# Autodesk Inventor assembly: Alliance Short Mogo
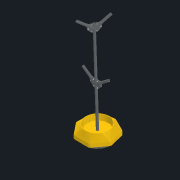
[picture p0: Inventor's stored thumbnail of the model, 180x180]
Saved by Autodesk Inventor 2021 (Build 250183000, 183)
## iProperties
Created: 2021-05-29
Part Number: Alliance Short Mogo
Document SubType Name: Assembly
Designer: max
Sending System: Autodesk Inventor 2021
Preprocessor: ST-DEVELOPER v18.1
Title: C:\Users\max\Desktop\Vex\TiP FieldCAD\Mogos\Alliance Short Mogo.stp
Author: max
Revision Number: ANY
## Documents named in this file (10)
- C:\Users\max\Desktop\Vex\TiP FieldCAD\Mogos\Alliance Tall Mogo.iam
- C:\Users\max\Desktop\Vex\TiP FieldCAD\Mogos\Screw 8-32 Steel .375.ipt
- C:\Users\max\Desktop\Vex\TiP FieldCAD\Mogos\Nut Nylock.ipt
- C:\Users\max\Desktop\Vex\TiP FieldCAD\Mogos\Mogo Branch Splitter.ipt
- C:\Users\max\Desktop\Vex\TiP FieldCAD\Mogos\Mogo Branch.ipt
- C:\Users\max\Desktop\Vex\TiP FieldCAD\Mogos\Mogo Post.ipt
- C:\Users\max\Desktop\Vex\TiP FieldCAD\Mogos\Mogo Base Post Grip.ipt
- C:\Users\max\Desktop\Vex\TiP FieldCAD\Mogos\Mogo Base Yellow.ipt
- C:\Users\max\Desktop\Vex\TiP FieldCAD\Mogos\Screw 8-32 Steel .625.ipt
- C:\Users\max\Desktop\Vex\TiP FieldCAD\Mogos\Mogo Base Bottom.ipt
## Components (45 placed, 9 different names)
1. Screw 8-32 Steel .375:1
2. Nut Nylock:1
3. Mogo Branch Splitter:1 — Angle:7
4. Mogo Branch:1
5. Mogo Post:1
6. Mogo Branch:2
7. Mogo Branch Splitter:2 — Mate:28, Mate:29
8. Screw 8-32 Steel .375:2
9. Nut Nylock:2
10. Screw 8-32 Steel .375:3
11. Nut Nylock:3
12. Screw 8-32 Steel .375:4
13. Nut Nylock:4
14. Screw 8-32 Steel .375:5
15. Nut Nylock:5
16. Screw 8-32 Steel .375:6
17. Nut Nylock:6
18. Mogo Base Post Grip:1
19. Mogo Base Yellow:1
20. Mogo Base Post Grip:2
21. Nut Nylock:7
22. Screw 8-32 Steel .625:7
23. Nut Nylock:8
24. Screw 8-32 Steel .625:8
25. Nut Nylock:9
26. Nut Nylock:10
27. Nut Nylock:11
28. Mogo Base Bottom:1
29. Mogo Branch Splitter:3 — Mate:8, Mate:9, Mate:10, Mate:11, Angle:7
30. Mogo Branch:3 — Mate:2, Mate:5
31. Mogo Post:2 — Mate:6, Mate:7, Mate:28, Mate:29
32. Mogo Branch:4 — Mate:3, Mate:4
33. Mogo Branch Splitter:4 — Mate:2, Mate:3, Mate:4, Mate:5, Mate:6, Mate:7, Mate:8, Mate:9, Mate:10, Mate:12, Mate:14, Mate:15, Mate:18, Mate:19, Mate:20, Mate:21, Mate:24, Mate:25, Angle:1, Angle:2, Mate:26, Mate:27, Angle:3, Angle:4, Angle:5, Angle:6
34. Screw 8-32 Steel .375:10 — Flush:1, Mate:1, Mate:11, Mate:12
35. Nut Nylock:15 — Flush:1, Mate:1, Angle:6
36. Screw 8-32 Steel .375:11 — Mate:14, Mate:15
37. Nut Nylock:16 — Angle:5
38. Screw 8-32 Steel .375:12 — Mate:18, Mate:20
39. Nut Nylock:17 — Angle:4
40. Screw 8-32 Steel .375:13 — Mate:19, Mate:21
41. Nut Nylock:18 — Angle:3
42. Screw 8-32 Steel .375:14 — Mate:26
43. Nut Nylock:19 — Mate:24, Angle:1
44. Screw 8-32 Steel .375:15 — Mate:27
45. Nut Nylock:20 — Mate:25, Angle:2
## Relationships (42: Mate 29, Angle 7, Flush 6)
- Flush:1 (-1.143 mm): Screw 8-32 Steel .375:10 ↔ Nut Nylock:15
- Mate:1: Screw 8-32 Steel .375:10 ↔ Nut Nylock:15
- Mate:2: Mogo Branch:3 ↔ Mogo Branch Splitter:4
- Mate:3: Mogo Branch:4 ↔ Mogo Branch Splitter:4
- Mate:4: Mogo Branch:4 ↔ Mogo Branch Splitter:4
- Mate:5: Mogo Branch:3 ↔ Mogo Branch Splitter:4
- Mate:6: Mogo Post:2 ↔ Mogo Branch Splitter:4
- Mate:7: Mogo Post:2 ↔ Mogo Branch Splitter:4
- Mate:8: Mogo Branch Splitter:3 ↔ Mogo Branch Splitter:4
- Mate:9: Mogo Branch Splitter:3 ↔ Mogo Branch Splitter:4
- Mate:10: Mogo Branch Splitter:3 ↔ Mogo Branch Splitter:4
- Mate:11: Mogo Branch Splitter:3 ↔ Screw 8-32 Steel .375:10
- Mate:12: Mogo Branch Splitter:4 ↔ Screw 8-32 Steel .375:10
- [Flush] (-1.143 mm): Screw 8-32 Steel .375:11 ↔ Nut Nylock:16
- [Mate]: Screw 8-32 Steel .375:11 ↔ Nut Nylock:16
- Mate:14: Mogo Branch Splitter:4 ↔ Screw 8-32 Steel .375:11
- Mate:15: Mogo Branch Splitter:4 ↔ Screw 8-32 Steel .375:11
- [Flush] (-1.143 mm): Screw 8-32 Steel .375:12 ↔ Nut Nylock:17
- [Mate]: Screw 8-32 Steel .375:12 ↔ Nut Nylock:17
- [Flush] (-1.143 mm): Screw 8-32 Steel .375:13 ↔ Nut Nylock:18
- [Mate]: Screw 8-32 Steel .375:13 ↔ Nut Nylock:18
- Mate:18: Mogo Branch Splitter:4 ↔ Screw 8-32 Steel .375:12
- Mate:19: Mogo Branch Splitter:4 ↔ Screw 8-32 Steel .375:13
- Mate:20: Mogo Branch Splitter:4 ↔ Screw 8-32 Steel .375:12
- Mate:21: Mogo Branch Splitter:4 ↔ Screw 8-32 Steel .375:13
- [Flush] (-1.143 mm): Screw 8-32 Steel .375:14 ↔ Nut Nylock:19
- [Mate]: Screw 8-32 Steel .375:14 ↔ Nut Nylock:19
- [Flush] (-1.143 mm): Screw 8-32 Steel .375:15 ↔ Nut Nylock:20
- [Mate]: Screw 8-32 Steel .375:15 ↔ Nut Nylock:20
- Mate:24: Mogo Branch Splitter:4 ↔ Nut Nylock:19
- Mate:25: Mogo Branch Splitter:4 ↔ Nut Nylock:20
- Angle:1 (0 deg): Mogo Branch Splitter:4 ↔ Nut Nylock:19
- Angle:2 (0 deg): Mogo Branch Splitter:4 ↔ Nut Nylock:20
- Mate:26: Mogo Branch Splitter:4 ↔ Screw 8-32 Steel .375:14
- Mate:27: Mogo Branch Splitter:4 ↔ Screw 8-32 Steel .375:15
- Angle:3 (0 deg): Mogo Branch Splitter:4 ↔ Nut Nylock:18
- Angle:4 (0 deg): Mogo Branch Splitter:4 ↔ Nut Nylock:17
- Angle:5 (0 deg): Mogo Branch Splitter:4 ↔ Nut Nylock:16
- Angle:6 (0 deg): Mogo Branch Splitter:4 ↔ Nut Nylock:15
- Mate:28: Mogo Branch Splitter:2 ↔ Mogo Post:2
- Mate:29: Mogo Branch Splitter:2 ↔ Mogo Post:2
- Angle:7 (5156.6202 deg): Mogo Branch Splitter:1 ↔ Mogo Branch Splitter:3
## Named parameters: d13_d0 = -1.143 mm, d14_d1 = 0 mm, d17_d13_d0 = -1.143 mm, d18_d14_d1 = 0 mm, d19_d13_d0 = -1.143 mm, d20_d14_d1 = 0 mm, d25_d13_d0 = -1.143 mm, d26_d14_d1 = 0 mm, d27_d13_d0 = -1.143 mm, d28_d14_d1 = 0 mm
